# Autodesk Inventor assembly: Board
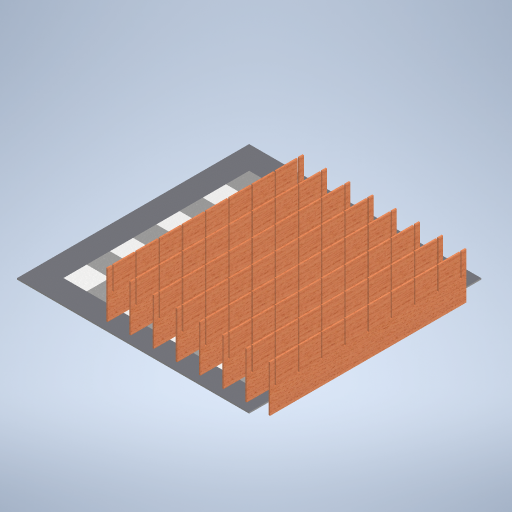
[picture p0: Inventor's stored thumbnail of the model, 512x512]
Saved by Autodesk Inventor 2024 (Build 280153000, 153)
## iProperties
Created: 2023-07-19
Part Number: Board
Document SubType Name: Assembly
Designer: Bruno
Author: Bruno
## Documents named in this file (3)
- D:\brucloud\utn\td2\proyecto\autodesk\Board.iam
- D:\brucloud\utn\td2\proyecto\autodesk\Board.ipt
- D:\brucloud\utn\td2\proyecto\autodesk\Separators.ipt
## Components (9 placed, 3 different names)
1. Board:1 — Flush:1
2. Separator — Flush:1
3. Separators:2
4. Separators:3
5. Separators:4
6. Separators:5
7. Separators:6
8. Separators:7
9. Separators:8
## Component patterns: (8 elements, first: Separator)
## Relationships (1: Flush 1)
- Flush:1: Board:1 ↔ Separator
